# Autodesk Inventor assembly: Gimble_stand
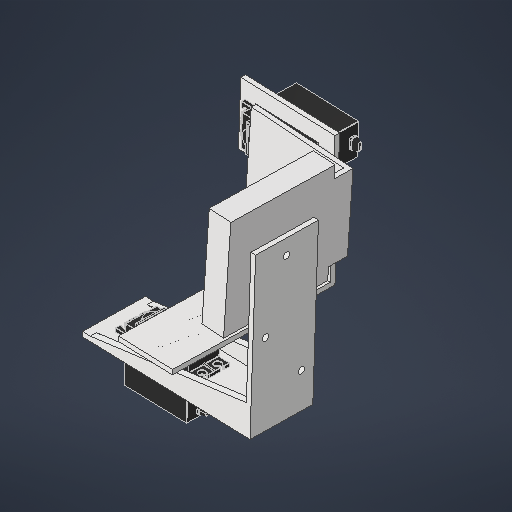
[picture p0: Inventor's stored thumbnail of the model, 512x512]
Saved by Autodesk Inventor 2026 (Build 300175000, 175)
## iProperties
Created: 2025-06-29
Part Number: Gimble_stand
Document SubType Name: Assembly
Designer: user
Author: user
## Documents named in this file (6)
- C:\Users\user\OneDrive - Ashesi University\third_year\System Engineering\Project\ping_pong_mechanism\Gimble_stand.iam
- C:\Users\user\OneDrive - Ashesi University\third_year\System Engineering\Project\ping_pong_mechanism\Servo Futaba S3003 v6\Servo Futaba S3003 v6\Part4.ipt
- C:\Users\user\OneDrive - Ashesi University\third_year\System Engineering\Project\ping_pong_mechanism\pan_base_holder_first.ipt
- C:\Users\user\OneDrive - Ashesi University\third_year\System Engineering\Project\ping_pong_mechanism\servo_motor_header.ipt
- C:\Users\user\OneDrive - Ashesi University\third_year\System Engineering\Project\ping_pong_mechanism\pan_base_holder_v1.ipt
- C:\Users\user\OneDrive - Ashesi University\third_year\System Engineering\Project\ping_pong_mechanism\pan_base_holder_third_v2.ipt
## Components (7 placed, 5 different names)
1. Part4:1 — Mate:2, Mate:3, Mate:4, Mate:5, Mate:6
2. pan_base_holder_first:1 — Mate:2, Mate:3, Mate:4
3. servo_motor_header:1 — Mate:5, Mate:6, Mate:7, Mate:8, Mate:9
4. pan_base_holder_v1:1 — Mate:7, Mate:8, Mate:9, Mate:10, Mate:11, Mate:12
5. Part4:2 — Mate:10, Mate:11, Mate:12, Mate:13, Mate:14
6. servo_motor_header:2 — Mate:13, Mate:14, Mate:15, Mate:16, Mate:17
7. pan_base_holder_third_v2:1 — Mate:15, Mate:16, Mate:17
## Relationships (16: Mate 16)
- Mate:2: Part4:1 ↔ pan_base_holder_first:1
- Mate:3 (0.5 mm): Part4:1 ↔ pan_base_holder_first:1
- Mate:4 (0.25 mm): Part4:1 ↔ pan_base_holder_first:1
- Mate:5: Part4:1 ↔ servo_motor_header:1
- Mate:6: Part4:1 ↔ servo_motor_header:1
- Mate:7: servo_motor_header:1 ↔ pan_base_holder_v1:1
- Mate:8: servo_motor_header:1 ↔ pan_base_holder_v1:1
- Mate:9: servo_motor_header:1 ↔ pan_base_holder_v1:1
- Mate:10: pan_base_holder_v1:1 ↔ Part4:2
- Mate:11 (0.5 mm): pan_base_holder_v1:1 ↔ Part4:2
- Mate:12 (0.25 mm): pan_base_holder_v1:1 ↔ Part4:2
- Mate:13: Part4:2 ↔ servo_motor_header:2
- Mate:14: Part4:2 ↔ servo_motor_header:2
- Mate:15: servo_motor_header:2 ↔ pan_base_holder_third_v2:1
- Mate:16: servo_motor_header:2 ↔ pan_base_holder_third_v2:1
- Mate:17: servo_motor_header:2 ↔ pan_base_holder_third_v2:1
